# Autodesk Inventor assembly: Mark 6 - Pnuematic Assembly
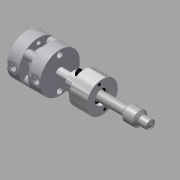
[picture p0: Inventor's stored thumbnail of the model, 180x180]
Saved by Autodesk Inventor 2013 (Build 170138000, 138)
## iProperties
Created: 2013-10-31
Part Number: Mark 6 - Pnuematic Assembly
Document SubType Name: Assembly
Designer: grtstudent
Author: grtstudent
## Documents named in this file (9)
- C:\Users\grtstudent\Desktop\Mark 6 Final Preseason\Mark 6 - Pnuematic Assembly.iam
- C:\Users\grtstudent\Desktop\Mark 6 Final Preseason\Pneumatic\Pancake Pneumatic.iam
- C:\Users\grtstudent\Desktop\Mark 6 Final Preseason\Pneumatic\Pneumatic Connector Cap.ipt
- C:\Users\grtstudent\Desktop\Mark 6 Final Preseason\Pneumatic\Pneumatic Connector.ipt
- C:\Users\grtstudent\Desktop\Mark 6 Final Preseason\Bolts\Socket Head Cap Screw 8-32 Thread .375 Length.ipt
- C:\Users\grtstudent\Desktop\Mark 6 Final Preseason\Shafts\Output Shaft\.0625 OD .25 Long Spring Pin.ipt
- C:\Users\grtstudent\Desktop\Mark 6 Final Preseason\Shafts\Output Shaft\Ball Shifting Shaft.ipt
- C:\Users\grtstudent\Desktop\Mark 6 Final Preseason\Bearings\R3-2RS.ipt
- C:\Users\grtstudent\Desktop\Mark 6 Final Preseason\Bolts\Socket Head Cap Screw 4-40 Thread .500 Length.ipt
## Components (9 placed, 8 different names)
1. Pancake Pneumatic:1 [sub-assembly] — Mate:1, Mate:2, Mate:14
2. Pneumatic Connector Cap:1 — Mate:11, Mate:12, Mate:13
3. Pneumatic Connector:1 — Mate:1, Mate:2, Mate:3, Mate:4, Mate:9, Mate:10, Mate:11, Mate:12, Mate:13, Mate:14, Mate:15, Mate:16, Mate:17, Mate:18
4. Socket Head Cap Screw 8-32 Thread .375 Length:1 — Mate:3, Mate:4
5. .0625 OD .25 Long Spring Pin:1 — Mate:5, Mate:6
6. Ball Shifting Shaft:1 — Mate:5, Mate:6, Mate:7, Mate:8
7. R3-2RS:1 — Mate:7, Mate:8, Mate:9, Mate:10
8. Socket Head Cap Screw 4-40 Thread .500 Length:1 — Mate:15, Mate:18
9. Socket Head Cap Screw 4-40 Thread .500 Length:2 — Mate:16, Mate:17
## Relationships (18: Mate 18)
- Mate:1: Pancake Pneumatic:1 ↔ Pneumatic Connector:1
- Mate:2: Pancake Pneumatic:1 ↔ Pneumatic Connector:1
- Mate:3: Pneumatic Connector:1 ↔ Socket Head Cap Screw 8-32 Thread .375 Length:1
- Mate:4: Pneumatic Connector:1 ↔ Socket Head Cap Screw 8-32 Thread .375 Length:1
- Mate:5: .0625 OD .25 Long Spring Pin:1 ↔ Ball Shifting Shaft:1
- Mate:6: .0625 OD .25 Long Spring Pin:1 ↔ Ball Shifting Shaft:1
- Mate:7: Ball Shifting Shaft:1 ↔ R3-2RS:1
- Mate:8: Ball Shifting Shaft:1 ↔ R3-2RS:1
- Mate:9: Pneumatic Connector:1 ↔ R3-2RS:1
- Mate:10: Pneumatic Connector:1 ↔ R3-2RS:1
- Mate:11: Pneumatic Connector Cap:1 ↔ Pneumatic Connector:1
- Mate:12: Pneumatic Connector Cap:1 ↔ Pneumatic Connector:1
- Mate:13: Pneumatic Connector Cap:1 ↔ Pneumatic Connector:1
- Mate:14: Pancake Pneumatic:1 ↔ Pneumatic Connector:1
- Mate:15: Pneumatic Connector:1 ↔ Socket Head Cap Screw 4-40 Thread .500 Length:1
- Mate:16: Pneumatic Connector:1 ↔ Socket Head Cap Screw 4-40 Thread .500 Length:2
- Mate:17: Pneumatic Connector:1 ↔ Socket Head Cap Screw 4-40 Thread .500 Length:2
- Mate:18: Pneumatic Connector:1 ↔ Socket Head Cap Screw 4-40 Thread .500 Length:1
